# Autodesk Inventor assembly: Cyberarm
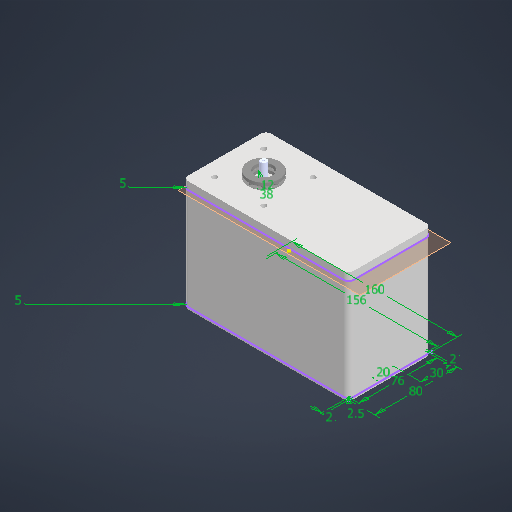
[picture p0: Inventor's stored thumbnail of the model, 512x512]
Saved by Autodesk Inventor 2026.1 (Build 301233020, 233B)
## iProperties
Created: 2025-10-18
Part Number: Cyberarm
Document SubType Name: Assembly
Designer: Nathan
Author: Nathan
## Documents named in this file (6)
- C:\Users\Nathan\Documents\GitHub\Cyberarm\hardware\cad\Cyberarm.iam
- C:\Users\Nathan\Documents\GitHub\Cyberarm\hardware\cad\Base.ipt
- C:\Users\Nathan\Documents\GitHub\Cyberarm\hardware\cad\BaseTop.ipt
- C:\Users\Nathan\Documents\GitHub\Cyberarm\hardware\cad\NEMA_23_57x76.ipt
- C:\Users\Nathan\Documents\GitHub\Cyberarm\hardware\cad\CXKG-1-D20-d6.35-e6.35\CXKG-1-D20-d6.35-e6.35\CXKG-1-D20-d6.35-e6.35.ipt
- C:\Users\Nathan\Documents\GitHub\Cyberarm\hardware\cad\BCTX-51103\BCTX-51103\BCTX-51103.ipt
## Components (5 placed, 5 different names)
1. Base:1
2. BaseTop:1 — Mate:1, Insert:1
3. NEMA_23_57x76:1 — Mate:1, Insert:2
4. CXKG-1-D20-d6.35-e6.35:1 — Insert:2
5. BCTX-51103:1 — Insert:1
## Relationships (3: Insert 2, Mate 1)
- Mate:1: BaseTop:1 ↔ NEMA_23_57x76:1
- Insert:1: BaseTop:1 ↔ BCTX-51103:1
- Insert:2 (-7 mm): NEMA_23_57x76:1 ↔ CXKG-1-D20-d6.35-e6.35:1
